# Autodesk Inventor assembly: Practica23.8
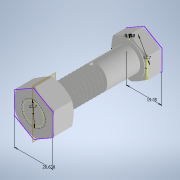
[picture p0: Inventor's stored thumbnail of the model, 180x180]
Saved by Autodesk Inventor 2020 (Build 240168000, 168)
## iProperties
Created: 2020-04-21
Part Number: Practica23.8
Document SubType Name: Assembly
Designer: luisg
Author: luisg
## Documents named in this file (3)
- C:\Users\luisg\Desktop\Examen Unidad I INVENTOR\Practica 23.8\Practica23.8.iam
- C:\Users\luisg\Desktop\Examen Unidad I INVENTOR\Practica 23.8\Practica2.3.8.1.ipt
- C:\Users\luisg\Desktop\Examen Unidad I INVENTOR\Practica 23.8\Practica2.3.8.2.ipt
## Components (2 placed, 2 different names)
1. Practica2.3.8.1:1 — Coincidencia:1
2. Practica2.3.8.2:1 — Coincidencia:1
## Relationships (1: Mate 1)
- Coincidencia:1 [Mate]: Practica2.3.8.1:1 ↔ Practica2.3.8.2:1
